# Autodesk Inventor assembly: Griber samlet_V1d
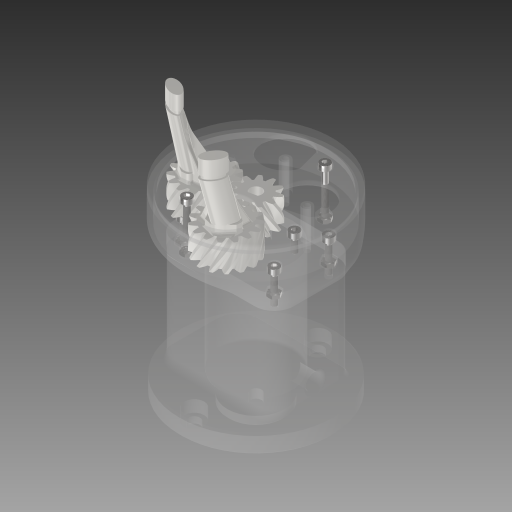
[picture p0: Inventor's stored thumbnail of the model, 512x512]
Saved by Autodesk Inventor 2024 (Build 280153000, 153)
## iProperties
Created: 2024-03-08
Part Number: Griber samlet_V1d
Document SubType Name: Assembly
Designer: Faber
Author: Faber
## Documents named in this file (10)
- C:\Users\Bluex\OneDrive - Syddansk Universitet\2. Semester\Semesterprojekt i autonome robotter\Inventor filer\Griber samlet_V1d.iam
- C:\Users\Bluex\OneDrive - Syddansk Universitet\2. Semester\Semesterprojekt i autonome robotter\Inventor filer\Motor_Hus_V1b.ipt
- C:\Users\Bluex\Documents\Inventor\Content Center Files\R2024\en-US\ISO 4032(1)\ISO 4032 - M3DIN EN.ipt
- C:\Users\Bluex\Documents\Inventor\Content Center Files\R2024\en-US\ISO 4762(1)\DIN EN ISO 4762 - M3 x 16.ipt
- C:\Users\Bluex\Documents\Inventor\Content Center Files\R2024\en-US\ISO 4762(1)\DIN EN ISO 4762 - M3 x 8.ipt
- C:\Users\Bluex\Documents\Inventor\Content Center Files\R2024\en-US\ISO 4762(1)\DIN EN ISO 4762 - M3 x 25.ipt
- C:\Users\Bluex\OneDrive - Syddansk Universitet\2. Semester\Semesterprojekt i autonome robotter\Inventor filer\Gear_Hus_V1d.ipt
- C:\Users\Bluex\OneDrive - Syddansk Universitet\2. Semester\Semesterprojekt i autonome robotter\Inventor filer\Gear_Assembly\Design Accelerator\Spur Gear11.ipt
- C:\Users\Bluex\OneDrive - Syddansk Universitet\2. Semester\Semesterprojekt i autonome robotter\Inventor filer\Gear_Assembly\Design Accelerator\Spur Gear21.ipt
- C:\Users\Bluex\OneDrive - Syddansk Universitet\2. Semester\Semesterprojekt i autonome robotter\Inventor filer\Gear_Hus_Laag_V1d.ipt
## Components (21 placed, 9 different names)
1. Motor_Hus_V1b:1 — Mate:16, Mate:17, Mate:18, Mate:19, Mate:20, Mate:21, Mate:22, Mate:23, Mate:24, Mate:25, Mate:26
2. DIN EN 24032 M3:1 — Mate:16, Mate:17, Mate:38
3. DIN EN 24032 M3:2 — Mate:18, Mate:19, Mate:41
4. DIN EN 24032 M3:3 — Mate:20, Mate:21, Mate:43
5. DIN EN 24032 M3:4 — Mate:22, Mate:23
6. DIN EN ISO 4762 M3 x 16:1 — Mate:40, Mate:41
7. DIN EN ISO 4762 M3 x 16:2 — Mate:42, Mate:43
8. DIN EN ISO 4762 M3 x 16:3 — Mate:38, Mate:39
9. DIN EN ISO 4762 M3 x 16:4 — Mate:31, Mate:49, Mate:64
10. DIN EN ISO 4762 M3 x 8:1 — Mate:36, Mate:37
11. DIN EN ISO 4762 M3 x 8:2 — Mate:32, Mate:33
12. DIN EN ISO 4762 M3 x 8:3 — Mate:34, Mate:35
13. DIN EN 24032 M3:6 — Mate:29, Mate:46
14. DIN EN ISO 4762 M3 x 25:1 — Mate:29, Mate:47, Mate:65
15. Gear_Hus_V1d:1 — Mate:24, Mate:25, Mate:26, Mate:32, Mate:33, Mate:34, Mate:35, Mate:36, Mate:37, Mate:39, Mate:40, Mate:42, Mate:46, Mate:47, Mate:48, Mate:49, Mate:53, Mate:54, Mate:55, Mate:56, Mate:57, Mate:58, Mate:59, Mate:60, Mate:61, Mate:62, Mate:63
16. DIN EN 24032 M3:8 — Mate:31, Mate:48
17. Spur Gear1:1 — Mate:53, Mate:58, Rotation:2, Rotation:3
18. Spur Gear2:1 — Mate:54, Mate:55, Rotation:2
19. Spur Gear2:2 — Mate:56, Mate:57, Rotation:3
20. Gear_Hus_Laag_V1d:1 — Mate:59, Mate:60, Mate:61, Mate:64, Mate:65
21. DIN EN ISO 4762 M3 x 16:5 — Mate:62, Mate:63
## Relationships (44: Mate 42, RelateRotation 2)
- Mate:16: Motor_Hus_V1b:1 ↔ DIN EN 24032 M3:1
- Mate:17: Motor_Hus_V1b:1 ↔ DIN EN 24032 M3:1
- Mate:18: Motor_Hus_V1b:1 ↔ DIN EN 24032 M3:2
- Mate:19: Motor_Hus_V1b:1 ↔ DIN EN 24032 M3:2
- Mate:20: Motor_Hus_V1b:1 ↔ DIN EN 24032 M3:3
- Mate:21: Motor_Hus_V1b:1 ↔ DIN EN 24032 M3:3
- Mate:22: Motor_Hus_V1b:1 ↔ DIN EN 24032 M3:4
- Mate:23: Motor_Hus_V1b:1 ↔ DIN EN 24032 M3:4
- Mate:24: Motor_Hus_V1b:1 ↔ Gear_Hus_V1d:1
- Mate:25: Motor_Hus_V1b:1 ↔ Gear_Hus_V1d:1
- Mate:26: Motor_Hus_V1b:1 ↔ Gear_Hus_V1d:1
- Mate:29: DIN EN 24032 M3:6 ↔ DIN EN ISO 4762 M3 x 25:1
- Mate:31: DIN EN ISO 4762 M3 x 16:4 ↔ DIN EN 24032 M3:8
- Mate:32: DIN EN ISO 4762 M3 x 8:2 ↔ Gear_Hus_V1d:1
- Mate:33: DIN EN ISO 4762 M3 x 8:2 ↔ Gear_Hus_V1d:1
- Mate:34: DIN EN ISO 4762 M3 x 8:3 ↔ Gear_Hus_V1d:1
- Mate:35: DIN EN ISO 4762 M3 x 8:3 ↔ Gear_Hus_V1d:1
- Mate:36: DIN EN ISO 4762 M3 x 8:1 ↔ Gear_Hus_V1d:1
- Mate:37: DIN EN ISO 4762 M3 x 8:1 ↔ Gear_Hus_V1d:1
- Mate:38: DIN EN 24032 M3:1 ↔ DIN EN ISO 4762 M3 x 16:3
- Mate:39: DIN EN ISO 4762 M3 x 16:3 ↔ Gear_Hus_V1d:1
- Mate:40: DIN EN ISO 4762 M3 x 16:1 ↔ Gear_Hus_V1d:1
- Mate:41: DIN EN 24032 M3:2 ↔ DIN EN ISO 4762 M3 x 16:1
- Mate:42: DIN EN ISO 4762 M3 x 16:2 ↔ Gear_Hus_V1d:1
- Mate:43: DIN EN 24032 M3:3 ↔ DIN EN ISO 4762 M3 x 16:2
- Mate:46: DIN EN 24032 M3:6 ↔ Gear_Hus_V1d:1
- Mate:47: DIN EN ISO 4762 M3 x 25:1 ↔ Gear_Hus_V1d:1
- Mate:48: Gear_Hus_V1d:1 ↔ DIN EN 24032 M3:8
- Mate:49: DIN EN ISO 4762 M3 x 16:4 ↔ Gear_Hus_V1d:1
- Mate:53: Gear_Hus_V1d:1 ↔ Spur Gear1:1
- Mate:54: Gear_Hus_V1d:1 ↔ Spur Gear2:1
- Mate:55: Gear_Hus_V1d:1 ↔ Spur Gear2:1
- Mate:56: Gear_Hus_V1d:1 ↔ Spur Gear2:2
- Mate:57: Gear_Hus_V1d:1 ↔ Spur Gear2:2
- Mate:58: Gear_Hus_V1d:1 ↔ Spur Gear1:1
- Rotation:2 [RelateRotation] (0.7333 ul): Spur Gear1:1 ↔ Spur Gear2:1
- Rotation:3 [RelateRotation] (0.7333 ul): Spur Gear1:1 ↔ Spur Gear2:2
- Mate:59: Gear_Hus_V1d:1 ↔ Gear_Hus_Laag_V1d:1
- Mate:60: Gear_Hus_V1d:1 ↔ Gear_Hus_Laag_V1d:1
- Mate:61: Gear_Hus_V1d:1 ↔ Gear_Hus_Laag_V1d:1
- Mate:62: Gear_Hus_V1d:1 ↔ DIN EN ISO 4762 M3 x 16:5
- Mate:63: Gear_Hus_V1d:1 ↔ DIN EN ISO 4762 M3 x 16:5
- Mate:64: DIN EN ISO 4762 M3 x 16:4 ↔ Gear_Hus_Laag_V1d:1
- Mate:65: DIN EN ISO 4762 M3 x 25:1 ↔ Gear_Hus_Laag_V1d:1
## Named parameters: Finish4_Area = 0.0396452
note: some values were not read from the file. Shown as the stored number, unit unknown: "Finish4_Area".
